# Autodesk Inventor assembly: Montagem
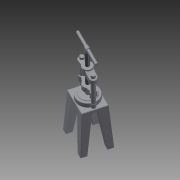
[picture p0: Inventor's stored thumbnail of the model, 180x180]
Saved by Autodesk Inventor 2015 (Build 190159000, 159)
## iProperties
Created: 2015-08-28
Part Number: Montagem
Document SubType Name: Assembly
Designer: EriveltonDell
Author: EriveltonDell
## Documents named in this file (6)
- C:\Users\EriveltonDell\Documents\Centro Universitário da FEI\8 ciclo\Elementos de Máquina II\Projeto\Balancim Manual\Montagem.iam
- C:\Users\EriveltonDell\Documents\Centro Universitário da FEI\8 ciclo\Elementos de Máquina II\Projeto\Balancim Manual\Base.ipt
- C:\Users\EriveltonDell\Documents\Centro Universitário da FEI\8 ciclo\Elementos de Máquina II\Projeto\Balancim Manual\Pino de Apoio.ipt
- C:\Users\EriveltonDell\Documents\Centro Universitário da FEI\8 ciclo\Elementos de Máquina II\Projeto\Balancim Manual\Base Superior.ipt
- C:\Users\EriveltonDell\Documents\Centro Universitário da FEI\8 ciclo\Elementos de Máquina II\Projeto\Balancim Manual\slide.ipt
- C:\Users\EriveltonDell\Documents\Centro Universitário da FEI\8 ciclo\Elementos de Máquina II\Projeto\Balancim Manual\fuso.ipt
## Components (6 placed, 5 different names)
1. Base:1 — Insert:1, Insert:2
2. Pino de Apoio:1 — Insert:1, Insert:3, Insert:4
3. Pino de Apoio:2 — Insert:2, Tangent:1
4. Base Superior:1 — Insert:3, Tangent:1, Insert:4, Insert:6
5. slide:1 — Insert:5
6. fuso:1 — Insert:5, Insert:6
## Relationships (7: Insert 6, Tangent 1)
- Insert:1: Base:1 ↔ Pino de Apoio:1
- Insert:2 (-50 mm): Base:1 ↔ Pino de Apoio:2
- Insert:3 (-70 mm): Pino de Apoio:1 ↔ Base Superior:1
- Tangent:1: Pino de Apoio:2 ↔ Base Superior:1
- Insert:4 (-130 mm): Pino de Apoio:1 ↔ Base Superior:1
- Insert:5 (-50 mm): slide:1 ↔ fuso:1
- Insert:6 (300 mm): Base Superior:1 ↔ fuso:1
